# Autodesk Inventor assembly: square_alt_assem
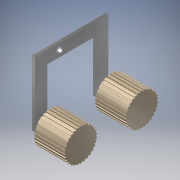
[picture p0: Inventor's stored thumbnail of the model, 180x180]
Saved by Autodesk Inventor 2018.1 (Build 221171000, 171)
## iProperties
Created: 2017-10-26
Part Number: square_alt_assem
Material: 一般
Document SubType Name: Assembly
Designer: Kakeru Yamashita
Author: Kakeru Yamashita
## Documents named in this file (3)
- C:\Users\Kakeru Yamashita\Documents\Inventor\Rocker_bogie_sim\square_alt_assem.iam
- C:\Users\Kakeru Yamashita\Documents\Inventor\Rocker_bogie_sim\bogie_square_alt.ipt
- C:\Users\Kakeru Yamashita\Documents\Inventor\Rocker_bogie_sim\tire.ipt
## Components (3 placed, 2 different names)
1. bogie_square_alt:1 — メイト:1, メイト:2, フラッシュ:2
2. tire:1 — メイト:2, フラッシュ:1
3. tire:2 — メイト:1, フラッシュ:1, フラッシュ:2
## Relationships (4: Mate 2, Flush 2)
- メイト:1 [Mate]: bogie_square_alt:1 ↔ tire:2
- メイト:2 [Mate]: bogie_square_alt:1 ↔ tire:1
- フラッシュ:1 [Flush]: tire:1 ↔ tire:2
- フラッシュ:2 [Flush]: bogie_square_alt:1 ↔ tire:2
